# Autodesk Inventor assembly: Fc Fender Assembly_MIR5
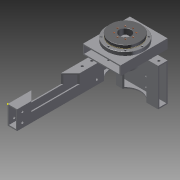
[picture p0: Inventor's stored thumbnail of the model, 180x180]
Saved by Autodesk Inventor 2015 (Build 190159000, 159)
## iProperties
Created: 2015-01-18
Part Number: Fc Fender Assembly_MIR5
Document SubType Name: Assembly
Designer: chapale16
Author: chapale16
## Documents named in this file (4)
- \\lhssvr02\Homedirs\Robotics Club\CAD Model 2015\Fc Fender Assembly_MIR5.iam
- \\lhssvr02\Homedirs\Robotics Club\CAD Model 2015\Alternate Arm mounts\BoxBeam and Igus Mount.iam
- \\lhssvr02\Homedirs\Robotics Club\CAD Model 2015\Alternate Arm mounts\Front Fender BoxBeam.ipt
- \\lhssvr02\Homedirs\Robotics Club\CAD Model 2015\Alternate Arm mounts\Fender Side Right.ipt
## Components (3 placed, 3 different names)
1. BoxBeam and Igus Mount:1 [sub-assembly]
2. Front Fender BoxBeam:1 — Flush:1, Mate:1, Flush:2
3. Fender Side Right:1 — Flush:1, Mate:1, Flush:2
## Relationships (3: Flush 2, Mate 1)
- Flush:1: Front Fender BoxBeam:1 ↔ Fender Side Right:1
- Mate:1: Front Fender BoxBeam:1 ↔ Fender Side Right:1
- Flush:2: Front Fender BoxBeam:1 ↔ Fender Side Right:1
